# Autodesk Inventor assembly: Assembly1
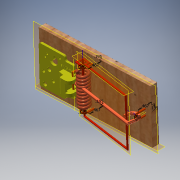
[picture p0: Inventor's stored thumbnail of the model, 180x180]
Saved by Autodesk Inventor 2016 (Build 200138000, 138)
## iProperties
Created: 2017-11-15
Part Number: Assembly1
Document SubType Name: Assembly
Designer: sun01147
Author: sun01147
## Documents named in this file (8)
- E:\IED7_SunT\IED7_MouseTrap\Assembly1.iam
- E:\IED7_SunT\IED7_MouseTrap\Sun_BaseStaple.ipt
- E:\IED7_SunT\IED7_MouseTrap\Sun_LargeStaple.ipt
- E:\IED7_SunT\IED7_MouseTrap\Sun_SmallStaple.ipt
- E:\IED7_SunT\IED7_MouseTrap\Sun_Hammer.ipt
- E:\IED7_SunT\IED7_MouseTrap\Sun_CatchLever.ipt
- E:\IED7_SunT\IED7_MouseTrap\Sun_Coil.ipt
- E:\IED7_SunT\IED7_MouseTrap\Catch (1).ipt
## Components (9 placed, 7 different names)
1. Sun_BaseStaple:1 — Insert:1, Insert:2, Insert:3, Insert:4, Mate:1, Mate:2, Mate:4, Mate:5, Flush:1, Angle:1
2. Sun_LargeStaple:1 — Insert:1, Mate:5
3. Sun_SmallStaple:1 — Insert:2, Mate:1, Mate:6, Mate:8
4. Sun_SmallStaple:2 — Insert:4, Mate:4
5. Sun_SmallStaple:3 — Insert:3, Mate:2
6. Sun_Hammer:1 — Mate:6, Mate:7, Mate:8, Mate:9, Flush:1, Angle:1
7. Sun_CatchLever:1
8. Sun_Coil:1 — Mate:7, Mate:9
9. Catch (1):1
## Relationships (14: Mate 8, Insert 4, Flush 1, Angle 1)
- Insert:1: Sun_BaseStaple:1 ↔ Sun_LargeStaple:1
- Insert:2: Sun_BaseStaple:1 ↔ Sun_SmallStaple:1
- Insert:3: Sun_BaseStaple:1 ↔ Sun_SmallStaple:3
- Insert:4: Sun_BaseStaple:1 ↔ Sun_SmallStaple:2
- Mate:1: Sun_BaseStaple:1 ↔ Sun_SmallStaple:1
- Mate:2: Sun_BaseStaple:1 ↔ Sun_SmallStaple:3
- Mate:4: Sun_BaseStaple:1 ↔ Sun_SmallStaple:2
- Mate:5: Sun_BaseStaple:1 ↔ Sun_LargeStaple:1
- Mate:6: Sun_SmallStaple:1 ↔ Sun_Hammer:1
- Mate:7: Sun_Hammer:1 ↔ Sun_Coil:1
- Mate:8: Sun_SmallStaple:1 ↔ Sun_Hammer:1
- Mate:9: Sun_Hammer:1 ↔ Sun_Coil:1
- Flush:1 (45.72 mm): Sun_BaseStaple:1 ↔ Sun_Hammer:1
- Angle:1 (10 deg): Sun_BaseStaple:1 ↔ Sun_Hammer:1
